# Autodesk Inventor assembly: Umlenkrolle
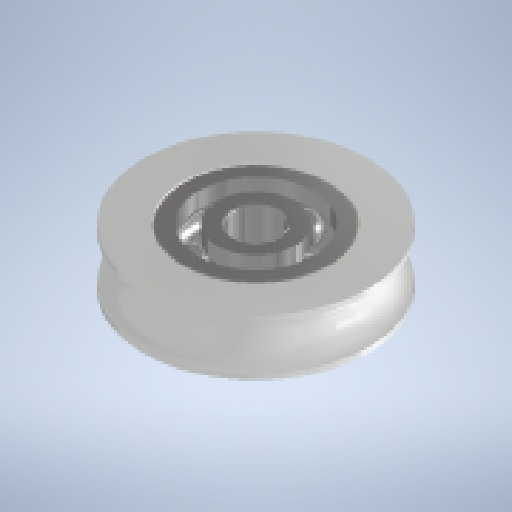
[picture p0: Inventor's stored thumbnail of the model, 512x512]
Saved by Autodesk Inventor 2025 (Build 290162010, 162A)
## iProperties
Created: 2024-11-18
Part Number: Umlenkrolle
Document SubType Name: Assembly
Designer: Admin
Mass: 3.73449 g
Surface Area: 17.7104 cm^2
Volume: 0.952055 cm^3
Density: 3.92255 g/cm^3
Author: Admin
## Documents named in this file (3)
- C:\Users\Admin\GIT\HDVKBM\CAD\Krandemonstrator\Umlenkrolle.iam
- C:\Users\Admin\GIT\HDVKBM\CAD\Krandemonstrator\Umlenkrolle\Konstruktions-Assistent\Lager1.iam
- C:\Users\Admin\GIT\HDVKBM\CAD\Krandemonstrator\Umlenkfläche.ipt
## Components (2 placed, 2 different names)
1. Lager:1 [sub-assembly] — Drehbar:1
2. Umlenkfläche:1 — Drehbar:1
## Relationships (1: RevoluteJoint 1)
- Drehbar:1 [RevoluteJoint]: Lager:1 ↔ Umlenkfläche:1
